# Autodesk Inventor assembly: COMPLETE_all_parts
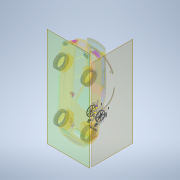
[picture p0: Inventor's stored thumbnail of the model, 180x180]
Saved by Autodesk Inventor 2021 (Build 250183000, 183)
## iProperties
Created: 2021-05-05
Part Number: COMPLETE_all_parts
Document SubType Name: Assembly
## Documents named in this file (4)
- C:\Users\ocon0143\OneDrive - Flinders\Advn Mech Design Shared\6_Development\2_Design\inventor\COMPLETE_all_parts.iam
- C:\Users\ocon0143\OneDrive - Flinders\Advn Mech Design Shared\6_Development\2_Design\inventor\cover\Assembly2.iam
- C:\Users\ocon0143\OneDrive - Flinders\Advn Mech Design Shared\6_Development\2_Design\inventor\hoop_slider\hoops_sml_med_lrg.iam
- C:\Users\ocon0143\OneDrive - Flinders\Advn Mech Design Shared\6_Development\2_Design\inventor\vehicle\mb_gls\ext_GLS Assembly.iam
## Components (3 placed, 3 different names)
1. Assembly2:1 [sub-assembly]
2. hoops_sml_med_lrg:1 [sub-assembly]
3. ext_GLS Assembly:1 [sub-assembly] — Flush:1, Mate:2
## Relationships (2: Flush 1, Mate 1)
- Flush:1: ext_GLS Assembly:1
- Mate:2 (-1600 mm): ext_GLS Assembly:1
